# Autodesk Inventor assembly: ProbeHead V3 - Assembly
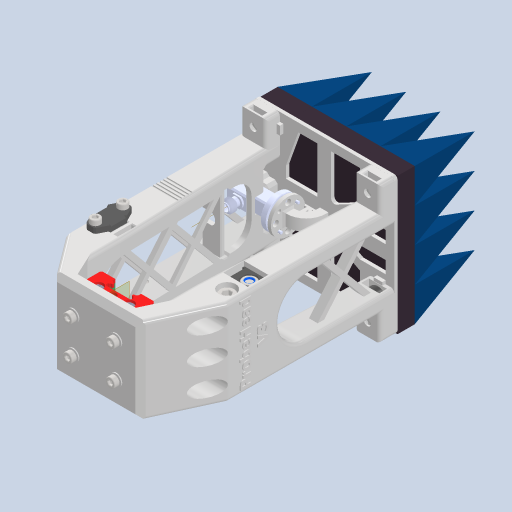
[picture p0: Inventor's stored thumbnail of the model, 512x512]
Saved by Autodesk Inventor 2023.2 (Build 272271000, 271)
## iProperties
Created: 2024-02-09
Part Number: ProbeHead V3 - Assembly
Document SubType Name: Assembly
Designer: Nils Bade
Author: Nils Bade
## Documents named in this file (17)
- C:\Users\nilsb\Documents\Inventor\Projektarbeit-Bade\RatRig_modified\ProbeHead\ProbeHead V3 - Assembly.iam
- C:\Users\nilsb\Documents\Inventor\Projektarbeit-Bade\RatRig_modified\MGN15 Linear-Rail-Block.ipt
- C:\Users\nilsb\Documents\Inventor\Projektarbeit-Bade\RatRig_Standards\face_belt_grabber v2.ipt
- C:\Users\nilsb\Documents\Inventor\Projektarbeit-Bade\Schrauben\Cap Head Screw M3x12 v2.ipt
- C:\Users\nilsb\Documents\Inventor\Projektarbeit-Bade\RatRig_Standards\Hex Nut - M3 v2.ipt
- C:\Users\nilsb\Documents\Inventor\Projektarbeit-Bade\Schrauben\Cap Head Screw M5x40 v2.ipt
- C:\Users\nilsb\Documents\Inventor\Projektarbeit-Bade\RatRig_Standards\Hex Locking Nut - M5 v2.ipt
- C:\Users\nilsb\Documents\Inventor\Projektarbeit-Bade\Schrauben\Washer Simple M3 - DIN6902.ipt
- C:\Users\nilsb\Documents\Inventor\Projektarbeit-Bade\RatRig_modified\ProbeHead\Wire2Probe_Eravant_SWC-15VF-R1-V.ipt
- C:\Users\nilsb\Documents\Inventor\Projektarbeit-Bade\Enclosure\Absorber\Absorber - IHF-Mini.ipt
- C:\Users\nilsb\Documents\Inventor\Projektarbeit-Bade\RatRig_modified\core_xy_belt_grabber_Bade.ipt
- C:\Users\nilsb\Documents\Inventor\Projektarbeit-Bade\RatRig_modified\ProbeHead\ProbeHead-Arms V3.ipt
- C:\Users\nilsb\Documents\Inventor\Projektarbeit-Bade\RatRig_modified\ProbeHead\ProbeAntennas\ProbeAntenna_V1.ipt
- C:\Users\nilsb\Documents\Inventor\Projektarbeit-Bade\RatRig_modified\ProbeHead\ProbeHead_Kabelfixieung_V1.ipt
- C:\Users\nilsb\Documents\Inventor\Projektarbeit-Bade\Enclosure\Magnet-RatrigEnclosure.ipt
- C:\Users\nilsb\Documents\Inventor\Projektarbeit-Bade\RatRig_Standards\Hex Nut - M4 DIN934.ipt
- C:\Users\nilsb\Documents\Inventor\Projektarbeit-Bade\Schrauben\Cap Head Screw M4x8 - DIN912.ipt
## Components (58 placed, 16 different names)
1. ProbeHead-Arms_V3:1 — Passend:62, Passend:63, Passend:64, Passend:67, Passend:70, Passend:71, Passend:72, Passend:73, Passend:74, Passend:75, Passend:76, Passend:77, Passend:78, Passend:79, Passend:80, Passend:81, Passend:82, Passend:83, Winkel:13, Winkel:14, Winkel:15, Winkel:16, Passend:84, Passend:85, Passend:86, Passend:87
2. core_xy_belt_grabber_Bade:2
3. core_xy_belt_grabber_Bade:1
4. MGN15 Linear-Rail-Block:1
5. face_belt_grabber v2:1 — Passend:16, Passend:17, Passend:18, Passend:19
6. face_belt_grabber v2:2 — Passend:12, Passend:13, Passend:14, Passend:15
7. Cap Head Screw M3x12 v2:1 — Passend:16, Passend:18, Passend:20
8. Cap Head Screw M3x12 v2:2 — Passend:17, Passend:19, Passend:21
9. Cap Head Screw M3x12 v2:3 — Passend:12, Passend:14, Passend:22
10. Cap Head Screw M3x12 v2:4 — Passend:13, Passend:15, Passend:23
11. Hex Nut - M3 v2:1 — Passend:20
12. Hex Nut - M3 v2:2 — Passend:23
13. Hex Nut - M3 v2:3 — Passend:22
14. Hex Nut - M3 v2:4 — Passend:21
15. Cap Head Screw M5x40 v2:1 — Passend:34
16. Cap Head Screw M5x40 v2:2
17. Hex Locking Nut - M5 v2:1
18. Hex Locking Nut - M5 v2:2 — Passend:34
19. Washer Simple M3 - DIN6902:1 — Passend:59
20. Washer Simple M3 - DIN6902:2 — Passend:56
21. Washer Simple M3 - DIN6902:3 — Passend:58
22. Washer Simple M3 - DIN6902:4 — Passend:57
23. Cap Head Screw M3x12 v2:5 — Passend:59
24. Cap Head Screw M3x12 v2:6 — Passend:58
25. Cap Head Screw M3x12 v2:7 — Passend:56
26. Cap Head Screw M3x12 v2:8 — Passend:57
27. Wire2Probe_Eravant_SWC-15VF-R1-V:1 — Passend:65, Winkel:12, Passend:66, Passend:68
28. ProbeAntenna V1:1 — Passend:62, Passend:63, Passend:64, Passend:65, Winkel:12, Passend:66, Fluchtend:3, Fluchtend:4, Passend:69, Passend:88, Passend:89, Passend:90, Passend:91, Passend:92, Passend:93, Passend:94, Passend:95
29. ProbeHead_Kabelfixieung_V1:1 — Passend:67, Passend:68
30. Magnet-RatrigEnclosure:1 — Passend:70, Passend:75
31. Magnet-RatrigEnclosure:2 — Passend:73, Passend:76
32. Magnet-RatrigEnclosure:3 — Passend:72, Passend:77
33. Magnet-RatrigEnclosure:4 — Passend:71, Passend:74
34. Magnet-RatrigEnclosure:5 — Passend:78, Passend:79
35. Hex Nut - M4 DIN934:1 — Passend:80, Winkel:13, Passend:87
36. Hex Nut - M4 DIN934:2 — Passend:81, Winkel:14, Passend:86
37. Hex Nut - M4 DIN934:3 — Passend:82, Winkel:15, Passend:85
38. Hex Nut - M4 DIN934:4 — Passend:83, Winkel:16, Passend:84
39. Cap Head Screw M4x8 - DIN912:1 — Passend:89, Passend:93
40. Cap Head Screw M4x8 - DIN912:2 — Passend:88, Passend:94
41. Cap Head Screw M4x8 - DIN912:3 — Passend:91, Passend:95
42. Cap Head Screw M4x8 - DIN912:4 — Passend:90, Passend:92
43. Absorber - IHF-Mini:1 — Fluchtend:3, Fluchtend:4, Passend:69
44. Absorber - IHF-Mini:2
45. Absorber - IHF-Mini:3
46. Absorber - IHF-Mini:4
47. Absorber - IHF-Mini:5
48. Absorber - IHF-Mini:6
49. Absorber - IHF-Mini:7
50. Absorber - IHF-Mini:8
51. Absorber - IHF-Mini:9
52. Absorber - IHF-Mini:10
53. Absorber - IHF-Mini:11
54. Absorber - IHF-Mini:12
55. Absorber - IHF-Mini:13
56. Absorber - IHF-Mini:14
57. Absorber - IHF-Mini:15
58. Absorber - IHF-Mini:16
## Component patterns: (16 elements, first: Absorber - IHF-Mini:1)
## Relationships (102: Mate 85, Angle 13, Flush 4)
- [Mate]: ProbeHead-Arms_V3:1 ↔ MGN15 Linear-Rail-Block:1
- [Mate]: ProbeHead-Arms_V3:1 ↔ MGN15 Linear-Rail-Block:1
- [Mate]: ProbeHead-Arms_V3:1 ↔ MGN15 Linear-Rail-Block:1
- [Mate]: ProbeHead-Arms_V3:1 ↔ core_xy_belt_grabber_Bade:1
- [Angle] (0 deg): ProbeHead-Arms_V3:1 ↔ core_xy_belt_grabber_Bade:2
- [Mate]: ProbeHead-Arms_V3:1 ↔ core_xy_belt_grabber_Bade:2
- [Flush] (2 mm): ProbeHead-Arms_V3:1 ↔ core_xy_belt_grabber_Bade:2
- [Flush] (2 mm): ProbeHead-Arms_V3:1 ↔ core_xy_belt_grabber_Bade:1
- [Mate]: ProbeHead-Arms_V3:1 ↔ face_belt_grabber v2:2
- [Mate]: ProbeHead-Arms_V3:1 ↔ face_belt_grabber v2:2
- [Mate]: ProbeHead-Arms_V3:1 ↔ face_belt_grabber v2:1
- [Mate]: ProbeHead-Arms_V3:1 ↔ face_belt_grabber v2:1
- Passend:12 [Mate]: face_belt_grabber v2:2 ↔ Cap Head Screw M3x12 v2:3
- Passend:13 [Mate]: face_belt_grabber v2:2 ↔ Cap Head Screw M3x12 v2:4
- Passend:14 [Mate]: face_belt_grabber v2:2 ↔ Cap Head Screw M3x12 v2:3
- Passend:15 [Mate]: face_belt_grabber v2:2 ↔ Cap Head Screw M3x12 v2:4
- Passend:16 [Mate]: face_belt_grabber v2:1 ↔ Cap Head Screw M3x12 v2:1
- Passend:17 [Mate]: face_belt_grabber v2:1 ↔ Cap Head Screw M3x12 v2:2
- Passend:18 [Mate]: face_belt_grabber v2:1 ↔ Cap Head Screw M3x12 v2:1
- Passend:19 [Mate]: face_belt_grabber v2:1 ↔ Cap Head Screw M3x12 v2:2
- Passend:20 [Mate]: Cap Head Screw M3x12 v2:1 ↔ Hex Nut - M3 v2:1
- Passend:21 [Mate]: Cap Head Screw M3x12 v2:2 ↔ Hex Nut - M3 v2:4
- Passend:22 [Mate]: Cap Head Screw M3x12 v2:3 ↔ Hex Nut - M3 v2:3
- Passend:23 [Mate]: Cap Head Screw M3x12 v2:4 ↔ Hex Nut - M3 v2:2
- [Angle] (0 deg): ProbeHead-Arms_V3:1 ↔ Hex Nut - M3 v2:1
- [Angle] (0 deg): ProbeHead-Arms_V3:1 ↔ Hex Nut - M3 v2:3
- [Mate]: ProbeHead-Arms_V3:1 ↔ Hex Nut - M3 v2:3
- [Mate]: ProbeHead-Arms_V3:1 ↔ Hex Nut - M3 v2:2
- [Mate]: ProbeHead-Arms_V3:1 ↔ Hex Nut - M3 v2:1
- [Mate]: ProbeHead-Arms_V3:1 ↔ Hex Nut - M3 v2:4
- [Mate]: ProbeHead-Arms_V3:1 ↔ Cap Head Screw M5x40 v2:2
- [Mate]: ProbeHead-Arms_V3:1 ↔ Cap Head Screw M5x40 v2:1
- [Mate]: ProbeHead-Arms_V3:1 ↔ Cap Head Screw M5x40 v2:1
- [Mate]: ProbeHead-Arms_V3:1 ↔ Cap Head Screw M5x40 v2:2
- [Mate]: core_xy_belt_grabber_Bade:1 ↔ Hex Locking Nut - M5 v2:1
- [Mate]: core_xy_belt_grabber_Bade:1 ↔ Hex Locking Nut - M5 v2:1
- Passend:34 [Mate]: Cap Head Screw M5x40 v2:1 ↔ Hex Locking Nut - M5 v2:2
- [Angle] (0 deg): core_xy_belt_grabber_Bade:2 ↔ Hex Locking Nut - M5 v2:2
- [Mate]: core_xy_belt_grabber_Bade:2 ↔ Hex Locking Nut - M5 v2:2
- [Angle] (0 deg): core_xy_belt_grabber_Bade:1 ↔ Hex Locking Nut - M5 v2:1
- [Mate]: ProbeHead-Arms_V3:1 ↔ Washer Simple M3 - DIN6902:1
- [Mate]: ProbeHead-Arms_V3:1 ↔ Washer Simple M3 - DIN6902:2
- [Mate]: ProbeHead-Arms_V3:1 ↔ Washer Simple M3 - DIN6902:3
- [Mate]: ProbeHead-Arms_V3:1 ↔ Washer Simple M3 - DIN6902:4
- [Mate]: ProbeHead-Arms_V3:1 ↔ Washer Simple M3 - DIN6902:4
- [Mate]: ProbeHead-Arms_V3:1 ↔ Washer Simple M3 - DIN6902:2
- [Mate]: ProbeHead-Arms_V3:1 ↔ Washer Simple M3 - DIN6902:1
- [Mate]: ProbeHead-Arms_V3:1 ↔ Washer Simple M3 - DIN6902:3
- [Mate]: ProbeHead-Arms_V3:1 ↔ Cap Head Screw M3x12 v2:5
- [Mate]: ProbeHead-Arms_V3:1 ↔ Cap Head Screw M3x12 v2:6
- [Mate]: ProbeHead-Arms_V3:1 ↔ Cap Head Screw M3x12 v2:7
- [Mate]: ProbeHead-Arms_V3:1 ↔ Cap Head Screw M3x12 v2:8
- Passend:56 [Mate]: Washer Simple M3 - DIN6902:2 ↔ Cap Head Screw M3x12 v2:7
- Passend:57 [Mate]: Washer Simple M3 - DIN6902:4 ↔ Cap Head Screw M3x12 v2:8
- Passend:58 [Mate]: Washer Simple M3 - DIN6902:3 ↔ Cap Head Screw M3x12 v2:6
- Passend:59 [Mate]: Washer Simple M3 - DIN6902:1 ↔ Cap Head Screw M3x12 v2:5
- [Mate]: ProbeHead-Arms_V3:1 ↔ Cap Head Screw M3x12 v2:4
- [Mate]: ProbeHead-Arms_V3:1 ↔ Cap Head Screw M3x12 v2:2
- [Angle] (0 deg): ProbeHead-Arms_V3:1 ↔ Hex Nut - M3 v2:2
- [Angle] (0 deg): ProbeHead-Arms_V3:1 ↔ Hex Nut - M3 v2:4
- [Angle] (180 deg): ProbeHead-Arms_V3:1 ↔ core_xy_belt_grabber_Bade:1
- Passend:62 [Mate]: ProbeHead-Arms_V3:1 ↔ ProbeAntenna V1:1
- Passend:63 [Mate]: ProbeHead-Arms_V3:1 ↔ ProbeAntenna V1:1
- Passend:64 [Mate]: ProbeHead-Arms_V3:1 ↔ ProbeAntenna V1:1
- Passend:65 [Mate]: Wire2Probe_Eravant_SWC-15VF-R1-V:1 ↔ ProbeAntenna V1:1
- Winkel:12 [Angle] (180 deg): Wire2Probe_Eravant_SWC-15VF-R1-V:1 ↔ ProbeAntenna V1:1
- Passend:66 [Mate]: Wire2Probe_Eravant_SWC-15VF-R1-V:1 ↔ ProbeAntenna V1:1
- Passend:67 [Mate]: ProbeHead-Arms_V3:1 ↔ ProbeHead_Kabelfixieung_V1:1
- Passend:68 [Mate]: Wire2Probe_Eravant_SWC-15VF-R1-V:1 ↔ ProbeHead_Kabelfixieung_V1:1
- Fluchtend:3 [Flush]: ProbeAntenna V1:1 ↔ Absorber - IHF-Mini:1
- Fluchtend:4 [Flush]: ProbeAntenna V1:1 ↔ Absorber - IHF-Mini:1
- Passend:69 [Mate]: ProbeAntenna V1:1 ↔ Absorber - IHF-Mini:1
- Passend:70 [Mate]: ProbeHead-Arms_V3:1 ↔ Magnet-RatrigEnclosure:1
- Passend:71 [Mate]: ProbeHead-Arms_V3:1 ↔ Magnet-RatrigEnclosure:4
- Passend:72 [Mate]: ProbeHead-Arms_V3:1 ↔ Magnet-RatrigEnclosure:3
- Passend:73 [Mate]: ProbeHead-Arms_V3:1 ↔ Magnet-RatrigEnclosure:2
- Passend:74 [Mate]: ProbeHead-Arms_V3:1 ↔ Magnet-RatrigEnclosure:4
- Passend:75 [Mate]: ProbeHead-Arms_V3:1 ↔ Magnet-RatrigEnclosure:1
- Passend:76 [Mate]: ProbeHead-Arms_V3:1 ↔ Magnet-RatrigEnclosure:2
- Passend:77 [Mate]: ProbeHead-Arms_V3:1 ↔ Magnet-RatrigEnclosure:3
- Passend:78 [Mate]: ProbeHead-Arms_V3:1 ↔ Magnet-RatrigEnclosure:5
- Passend:79 [Mate]: ProbeHead-Arms_V3:1 ↔ Magnet-RatrigEnclosure:5
- Passend:80 [Mate]: ProbeHead-Arms_V3:1 ↔ Hex Nut - M4 DIN934:1
- Passend:81 [Mate]: ProbeHead-Arms_V3:1 ↔ Hex Nut - M4 DIN934:2
- Passend:82 [Mate]: ProbeHead-Arms_V3:1 ↔ Hex Nut - M4 DIN934:3
- Passend:83 [Mate]: ProbeHead-Arms_V3:1 ↔ Hex Nut - M4 DIN934:4
- Winkel:13 [Angle] (0 deg): ProbeHead-Arms_V3:1 ↔ Hex Nut - M4 DIN934:1
- Winkel:14 [Angle] (0 deg): ProbeHead-Arms_V3:1 ↔ Hex Nut - M4 DIN934:2
- Winkel:15 [Angle] (0 deg): ProbeHead-Arms_V3:1 ↔ Hex Nut - M4 DIN934:3
- Winkel:16 [Angle] (0 deg): ProbeHead-Arms_V3:1 ↔ Hex Nut - M4 DIN934:4
- Passend:84 [Mate]: ProbeHead-Arms_V3:1 ↔ Hex Nut - M4 DIN934:4
- Passend:85 [Mate]: ProbeHead-Arms_V3:1 ↔ Hex Nut - M4 DIN934:3
- Passend:86 [Mate]: ProbeHead-Arms_V3:1 ↔ Hex Nut - M4 DIN934:2
- Passend:87 [Mate]: ProbeHead-Arms_V3:1 ↔ Hex Nut - M4 DIN934:1
- Passend:88 [Mate]: ProbeAntenna V1:1 ↔ Cap Head Screw M4x8 - DIN912:2
- Passend:89 [Mate]: ProbeAntenna V1:1 ↔ Cap Head Screw M4x8 - DIN912:1
- Passend:90 [Mate]: ProbeAntenna V1:1 ↔ Cap Head Screw M4x8 - DIN912:4
- Passend:91 [Mate]: ProbeAntenna V1:1 ↔ Cap Head Screw M4x8 - DIN912:3
- Passend:92 [Mate]: ProbeAntenna V1:1 ↔ Cap Head Screw M4x8 - DIN912:4
- Passend:93 [Mate]: ProbeAntenna V1:1 ↔ Cap Head Screw M4x8 - DIN912:1
- Passend:94 [Mate]: ProbeAntenna V1:1 ↔ Cap Head Screw M4x8 - DIN912:2
- Passend:95 [Mate]: ProbeAntenna V1:1 ↔ Cap Head Screw M4x8 - DIN912:3
